# Autodesk Inventor assembly: chip
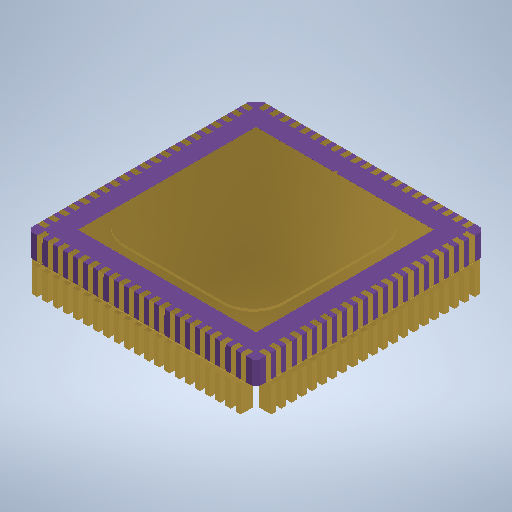
[picture p0: Inventor's stored thumbnail of the model, 512x512]
Saved by Autodesk Inventor 2025 (Build 290162000, 162)
## iProperties
Created: 2025-09-08
Part Number: chip
Document SubType Name: Assembly
Designer: jirne
Author: jirne
## Documents named in this file (4)
- C:\Users\jirne\JVR11\hardware\library\3D\DCJ11\chip\chip.iam
- C:\Users\jirne\JVR11\hardware\library\3D\DCJ11\chip\chip_body.ipt
- C:\Users\jirne\JVR11\hardware\library\3D\DCJ11\chip\plate.ipt
- C:\Users\jirne\JVR11\hardware\library\3D\DCJ11\chip\pins.ipt
## Components (86 placed, 3 different names)
1. chip_body:1 — Rigid:1, Mate:1, Mate:2, Mate:3, Mate:4, Mate:5, Mate:6, Mate:7, Mate:8
2. plate:1 — Rigid:1
3. pins:1 — Mate:1, Mate:2
4. pins:2
5. pins:3
6. pins:4
7. pins:5
8. pins:6
9. pins:7
10. pins:8
11. pins:9
12. pins:10
13. pins:11
14. pins:12
15. pins:13
16. pins:14
17. pins:15
18. pins:16
19. pins:17
20. pins:18
21. pins:19
22. pins:20
23. pins:21
24. pins:22 — Mate:3, Mate:4
25. pins:23
26. pins:24
27. pins:25
28. pins:26
29. pins:27
30. pins:28
31. pins:29
32. pins:30
33. pins:31
34. pins:32
35. pins:33
36. pins:34
37. pins:35
38. pins:36
39. pins:37
40. pins:38
41. pins:39
42. pins:40
43. pins:41
44. pins:42
45. pins:43 — Mate:5, Mate:6
46. pins:44
47. pins:45
48. pins:46
49. pins:47
50. pins:48
51. pins:49
52. pins:50
53. pins:51
54. pins:52
55. pins:53
56. pins:54
57. pins:55
58. pins:56
59. pins:57
60. pins:58
61. pins:59
62. pins:60
63. pins:61
64. pins:62
65. pins:63
66. pins:64 — Mate:7, Mate:8
67. pins:65
68. pins:66
69. pins:67
70. pins:68
71. pins:69
72. pins:70
73. pins:71
74. pins:72
75. pins:73
76. pins:74
77. pins:75
78. pins:76
79. pins:77
80. pins:78
81. pins:79
82. pins:80
83. pins:81
84. pins:82
85. pins:83
86. pins:84
## Component patterns: (21 elements, first: pins:1), (21 elements, first: pins:22), (21 elements, first: pins:43), (21 elements, first: pins:64)
## Relationships (9: Mate 8, WeldJoint 1)
- Rigid:1 [WeldJoint]: chip_body:1 ↔ plate:1
- Mate:1: chip_body:1 ↔ pins:1
- Mate:2: chip_body:1 ↔ pins:1
- Mate:3: chip_body:1 ↔ pins:22
- Mate:4: chip_body:1 ↔ pins:22
- Mate:5: chip_body:1 ↔ pins:43
- Mate:6: chip_body:1 ↔ pins:43
- Mate:7: chip_body:1 ↔ pins:64
- Mate:8: chip_body:1 ↔ pins:64
